# Autodesk Inventor assembly: +XPanel
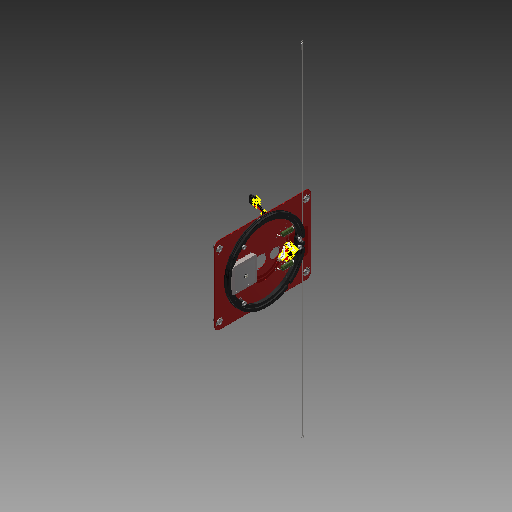
[picture p0: Inventor's stored thumbnail of the model, 512x512]
Saved by Autodesk Inventor 2018 (Build 220112000, 112)
## iProperties
Created: 2018-07-05
Part Number: +XPanel
Document SubType Name: Assembly
Designer: Bradley
Mass: 19.8214 g
Surface Area: 182.188 cm^2
Volume: 10.2774 cm^3
Density: 1.92865 g/cm^3
Author: Bradley
## Documents named in this file (18)
- D:\Users\Bradley\Documents\CougsInSpace\CougSat1-Hardware\CougSat1-AvionicBoard\CADModel\Native\+XPanel.iam
- D:\Users\Bradley\Documents\CougsInSpace\CougSat1-Hardware\CougSat1-AvionicBoard\CADModel\Native\+XPanel_PCB.ipt
- D:\Users\Bradley\Documents\CougsInSpace\Resources\ComponentModels\Electronics\Antenna_GPSPatch.ipt
- D:\Users\Bradley\Documents\CougsInSpace\Resources\ComponentModels\Fasteners\Bolt_M3x0.35_5mm_BH.ipt
- D:\Users\Bradley\Documents\CougsInSpace\CougSat1-Hardware\CougSat1-AvionicBoard\CADModel\Native\+XPanel_AntennaDeployed.ipt
- D:\Users\Bradley\Documents\CougsInSpace\CougSat1-Hardware\CougSat1-AvionicBoard\CADModel\Native\+XPanel_AntennaMount.ipt
- D:\Users\Bradley\Documents\CougsInSpace\Resources\ComponentModels\Fasteners\Bolt_M2x0.4_6mm_SH.ipt
- D:\Users\Bradley\Documents\CougsInSpace\Resources\ComponentModels\Electronics\Resistor_TH-15mm.ipt
- D:\Users\Bradley\Documents\CougsInSpace\CougSat1-Hardware\CougSat1-AvionicBoard\CADModel\Native\+XPanel_AntennaForm.ipt
- D:\Users\Bradley\Documents\CougsInSpace\Resources\ComponentModels\Connectors\PinRecepticle-0.38-0.56mm.ipt
- D:\Users\Bradley\Documents\CougsInSpace\CougSat1-Hardware\CougSat1-AvionicBoard\CADModel\Native\+XPanel_AntennaStowed+Y.ipt
- D:\Users\Bradley\Documents\CougsInSpace\CougSat1-Hardware\CougSat1-AvionicBoard\CADModel\Native\+XPanel_AntennaStowed-Y.ipt
- D:\Users\Bradley\Documents\CougsInSpace\CougSat1-Hardware\CougSat1-AvionicBoard\CADModel\Native\+XPanel_AntennaLine+Y.ipt
- D:\Users\Bradley\Documents\CougsInSpace\CougSat1-Hardware\CougSat1-AvionicBoard\CADModel\Native\+XPanel_AntennaLine-Y.ipt
- D:\Users\Bradley\Documents\CougsInSpace\Resources\ComponentModels\Connectors\PicoLock-P-4.ipt
- D:\Users\Bradley\Documents\CougsInSpace\CougSat1-Hardware\CougSat1-AvionicBoard\CADModel\Native\+XPanel\AIP\Cable and Harness\+XPanel.Harness1.iam
- D:\Users\Bradley\Documents\CougsInSpace\Resources\ComponentModels\Connectors\U.FL_Male.ipt
- D:\Users\Bradley\Documents\CougsInSpace\Resources\ComponentModels\Connectors\U.FL_Female.ipt
## Components (30 placed, 17 different names)
1. +XPanel_AntennaDeployed:1 — Mate:1, Mate:2
2. +XPanel_AntennaDeployed:2 — Mate:3, Mate:4
3. +XPanel_AntennaForm:1 — Insert:25, Insert:26, Insert:27, Insert:28, Insert:29, Insert:30, Insert:31
4. +XPanel_AntennaLine+Y:1 — Flush:2, Mate:10, Flush:3
5. +XPanel_AntennaLine-Y:1 — Flush:4, Mate:11, Flush:5
6. +XPanel_AntennaMount:1 — Mate:1, Mate:4, Insert:18, Insert:19, Insert:25, Insert:27, Mate:7, Mate:9
7. +XPanel_AntennaStowed+Y:1 — Mate:6, Mate:7
8. +XPanel_AntennaStowed-Y:1 — Mate:8, Mate:9
9. +XPanel_PCB:1 — Insert:1, Insert:2, Insert:3, Insert:4, Insert:5, Mate:2, Mate:3, Insert:20, Insert:21, Insert:22, Insert:23, Insert:26, Insert:28, Insert:29, Insert:32, Insert:33, Mate:6, Mate:8, Mate:13, Mate:14, Mate:15, Mate:16, Mate:17, Mate:18, Mate:19, Mate:20, Mate:21, Mate:22, Mate:23, Mate:24, Angle:3, Angle:4
10. Harness1 [sub-assembly]
11. PicoLock-P-4:1 — Mate:12, Flush:6, Flush:7
12. PinRecepticle-0.38-0.56mm:1 — Insert:33
13. PinRecepticle-0.38-0.56mm:2 — Insert:32
14. U.FL_Male:1 — Insert:34, Mate:13, Mate:14, Mate:15, Mate:16, Angle:1
15. U.FL_Male:2 — Mate:17, Mate:18, Mate:19, Mate:20, Angle:2
16. U.FL_Female:1 — Insert:34, Angle:1
17. U.FL_Female:2 — Angle:2
18. U.FL_Female:3 — Mate:21, Mate:22, Angle:3
19. U.FL_Female:4 — Mate:23, Mate:24, Angle:4
20. Antenna_GPSPatch:1 — Flush:1, Insert:1
21. Resistor_TH-15mm:1 — Insert:20, Insert:21, Mate:11
22. Resistor_TH-15mm:2 — Insert:22, Insert:23, Mate:10
23. Bolt_M2x0.4_6mm_SH:1 — Insert:30
24. Bolt_M2x0.4_6mm_SH:2 — Insert:31
25. Bolt_M2x0.4_6mm_SH:3 — Insert:19
26. Bolt_M2x0.4_6mm_SH:4 — Insert:18
27. Bolt_M3x0.35_5mm_BH:1 — Insert:2
28. Bolt_M3x0.35_5mm_BH:2 — Insert:3
29. Bolt_M3x0.35_5mm_BH:3 — Insert:4
30. Bolt_M3x0.35_5mm_BH:4 — Insert:5
## Relationships (56: Mate 23, Insert 22, Flush 7, Angle 4)
- Flush:1: Antenna_GPSPatch:1
- Insert:1: +XPanel_PCB:1 ↔ Antenna_GPSPatch:1
- Insert:2: +XPanel_PCB:1 ↔ Bolt_M3x0.35_5mm_BH:1
- Insert:3: +XPanel_PCB:1 ↔ Bolt_M3x0.35_5mm_BH:2
- Insert:4: +XPanel_PCB:1 ↔ Bolt_M3x0.35_5mm_BH:3
- Insert:5: +XPanel_PCB:1 ↔ Bolt_M3x0.35_5mm_BH:4
- Mate:1: +XPanel_AntennaDeployed:1 ↔ +XPanel_AntennaMount:1
- Mate:2: +XPanel_AntennaDeployed:1 ↔ +XPanel_PCB:1
- Mate:3: +XPanel_AntennaDeployed:2 ↔ +XPanel_PCB:1
- Mate:4: +XPanel_AntennaDeployed:2 ↔ +XPanel_AntennaMount:1
- Insert:18: +XPanel_AntennaMount:1 ↔ Bolt_M2x0.4_6mm_SH:4
- Insert:19: +XPanel_AntennaMount:1 ↔ Bolt_M2x0.4_6mm_SH:3
- Insert:20 (-1.235 mm): +XPanel_PCB:1 ↔ Resistor_TH-15mm:1
- Insert:21 (-1.235 mm): +XPanel_PCB:1 ↔ Resistor_TH-15mm:1
- Insert:22 (-1.235 mm): +XPanel_PCB:1 ↔ Resistor_TH-15mm:2
- Insert:23 (-1.235 mm): +XPanel_PCB:1 ↔ Resistor_TH-15mm:2
- Insert:25: +XPanel_AntennaForm:1 ↔ +XPanel_AntennaMount:1
- Insert:26: +XPanel_AntennaForm:1 ↔ +XPanel_PCB:1
- Insert:27: +XPanel_AntennaForm:1 ↔ +XPanel_AntennaMount:1
- Insert:28: +XPanel_AntennaForm:1 ↔ +XPanel_PCB:1
- Insert:29: +XPanel_AntennaForm:1 ↔ +XPanel_PCB:1
- Insert:30: +XPanel_AntennaForm:1 ↔ Bolt_M2x0.4_6mm_SH:1
- Insert:31: +XPanel_AntennaForm:1 ↔ Bolt_M2x0.4_6mm_SH:2
- Insert:32: +XPanel_PCB:1 ↔ PinRecepticle-0.38-0.56mm:2
- Insert:33: +XPanel_PCB:1 ↔ PinRecepticle-0.38-0.56mm:1
- Mate:6: +XPanel_AntennaStowed+Y:1 ↔ +XPanel_PCB:1
- Mate:7: +XPanel_AntennaMount:1 ↔ +XPanel_AntennaStowed+Y:1
- Mate:8: +XPanel_AntennaStowed-Y:1 ↔ +XPanel_PCB:1
- Mate:9: +XPanel_AntennaMount:1 ↔ +XPanel_AntennaStowed-Y:1
- Flush:2 (22 mm): +XPanel_AntennaLine+Y:1
- Mate:10: +XPanel_AntennaLine+Y:1 ↔ Resistor_TH-15mm:2
- Flush:3: +XPanel_AntennaLine+Y:1
- Flush:4 (21.65 mm): +XPanel_AntennaLine-Y:1
- Mate:11: +XPanel_AntennaLine-Y:1 ↔ Resistor_TH-15mm:1
- Flush:5: +XPanel_AntennaLine-Y:1
- Mate:12 (39 mm): PicoLock-P-4:1
- Flush:6 (-8.955 mm): PicoLock-P-4:1
- Flush:7 (-18.75 mm): PicoLock-P-4:1
- Insert:34 (0.1 mm): U.FL_Male:1 ↔ U.FL_Female:1
- Mate:13: +XPanel_PCB:1 ↔ U.FL_Male:1
- Mate:14: +XPanel_PCB:1 ↔ U.FL_Male:1
- Mate:15: +XPanel_PCB:1 ↔ U.FL_Male:1
- Mate:16: +XPanel_PCB:1 ↔ U.FL_Male:1
- [Insert] (0.1 mm): U.FL_Male:2 ↔ U.FL_Female:2
- Mate:17: +XPanel_PCB:1 ↔ U.FL_Male:2
- Mate:18: +XPanel_PCB:1 ↔ U.FL_Male:2
- Mate:19: +XPanel_PCB:1 ↔ U.FL_Male:2
- Mate:20: +XPanel_PCB:1 ↔ U.FL_Male:2
- Angle:1 (-5.88 deg): U.FL_Male:1 ↔ U.FL_Female:1
- Angle:2 (8.34 deg): U.FL_Male:2 ↔ U.FL_Female:2
- Mate:21: +XPanel_PCB:1 ↔ U.FL_Female:3
- Mate:22: +XPanel_PCB:1 ↔ U.FL_Female:3
- Mate:23: +XPanel_PCB:1 ↔ U.FL_Female:4
- Mate:24: +XPanel_PCB:1 ↔ U.FL_Female:4
- Angle:3 (7.43 deg): +XPanel_PCB:1 ↔ U.FL_Female:3
- Angle:4 (5.16 deg): +XPanel_PCB:1 ↔ U.FL_Female:4
## Named parameters: d66_d61 = 0.1 mm
